# Autodesk Inventor assembly: DrumCam
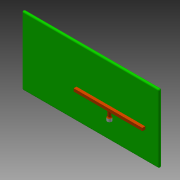
[picture p0: Inventor's stored thumbnail of the model, 180x180]
Saved by Autodesk Inventor 2015 (Build 190159000, 159)
## iProperties
Created: 2015-04-20
Part Number: DrumCam
Document SubType Name: Assembly
Designer: WASHHSST
Author: WASHHSST
## Documents named in this file (3)
- C:\Users\washhsst\Documents\GitHub\myWork\DrumCam_JacobMorgan_042015_pd3\DrumCam.iam
- C:\Users\washhsst\Documents\GitHub\myWork\DrumCam_JacobMorgan_042015_pd3\BasePlate.ipt
- C:\Users\washhsst\Documents\GitHub\myWork\DrumCam_JacobMorgan_042015_pd3\SquareTubeSlider.ipt
## Components (2 placed, 2 different names)
1. BasePlate:1 — Flush:1
2. SquareTubeSlider:1 — Flush:1
## Relationships (1: Flush 1)
- Flush:1: BasePlate:1 ↔ SquareTubeSlider:1
